# Autodesk Inventor assembly: Set
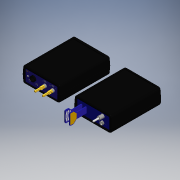
[picture p0: Inventor's stored thumbnail of the model, 180x180]
Saved by Autodesk Inventor 2016 (Build 200138000, 138)
## iProperties
Created: 2016-12-24
Part Number: Set
Document SubType Name: Assembly
Designer: Tyler
Author: Tyler
## Documents named in this file (3)
- C:\Users\Tyler\Documents\Small Projects\Personal\morse-practice-oscillator\Mechanicial\Set.iam
- C:\Users\Tyler\Documents\Small Projects\Personal\morse-practice-oscillator\Mechanicial\Sounder\Sounder.iam
- C:\Users\Tyler\Documents\Small Projects\Personal\morse-practice-oscillator\Mechanicial\Key\TouchKeyer.iam
## Components (2 placed, 2 different names)
1. Sounder:1 [sub-assembly] — Mate:1, Flush:2, Mate:2, Flush:3
2. TouchKeyer:1 [sub-assembly] — Flush:2, Mate:2, Flush:3
## Relationships (4: Mate 2, Flush 2)
- Mate:1: Sounder:1
- Flush:2: Sounder:1 ↔ TouchKeyer:1
- Mate:2 (25.4 mm): Sounder:1 ↔ TouchKeyer:1
- Flush:3: Sounder:1 ↔ TouchKeyer:1
